# Autodesk Inventor assembly: Wheel Vexpro 4in
Saved by Autodesk Inventor 2013 (Build 170138000, 138)
## iProperties
Created: 2014-07-12
Part Number: Wheel Vexpro 4in
Document SubType Name: Assembly
Designer: admin
Author: admin
## Documents named in this file (3)
- C:\Users\admin\Documents\GitHub\CAD\west coast drive\Wheel Vexpro 4in .iam
- C:\Users\admin\Documents\GitHub\2013-2014_BlockParty\CAD\COTSParts\Wheels\VexPro Traction Wheels\Components\Traction Tire Body 4in.ipt
- C:\Users\admin\Documents\GitHub\2013-2014_BlockParty\CAD\COTSParts\Hubs\VersaHub 500 Hex.ipt
## Components (4 placed, 2 different names)
1. Traction Tire Body 4in:1
2. Traction Tire Body 4in:2
3. VersaHub 500 Hex:1
4. VersaHub 500 Hex:2
## Relationships (10: Mate 10)
- [Mate]: Traction Tire Body 4in:1 ↔ Traction Tire Body 4in:2
- [Mate]: Traction Tire Body 4in:1 ↔ Traction Tire Body 4in:2
- [Mate]: Traction Tire Body 4in:1 ↔ Traction Tire Body 4in:2
- [Mate]: Traction Tire Body 4in:2 ↔ VersaHub 500 Hex:2
- [Mate]: Traction Tire Body 4in:2 ↔ VersaHub 500 Hex:2
- [Mate]: Traction Tire Body 4in:1 ↔ VersaHub 500 Hex:1
- [Mate]: Traction Tire Body 4in:1 ↔ VersaHub 500 Hex:1
- [Mate]: Traction Tire Body 4in:1 ↔ VersaHub 500 Hex:1
- [Mate]: Traction Tire Body 4in:2 ↔ VersaHub 500 Hex:2
- [Mate]: Traction Tire Body 4in:2 ↔ VersaHub 500 Hex:2
## Named parameters: d0_d2 = 0 mm, d1_d3 = 0 mm, d2_d4 = 0 mm, d3_d5 = 0 mm, d4_d6 = 0 mm, d5_d7 = 0 mm, d6_d8 = 0 mm, d7_d9 = 0 mm
